# Autodesk Inventor assembly: Baugruppe1
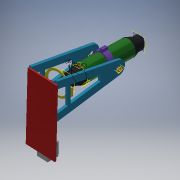
[picture p0: Inventor's stored thumbnail of the model, 180x180]
Saved by Autodesk Inventor 2017 (Build 210142000, 142)
## iProperties
Part Number: Baugruppe1
Material: Generisch
Document SubType Name: Assembly
Designer: Fabio
Author: Fabio
## Documents named in this file (10)
- C:\Users\Fabio\dicer\inventor\Baugruppe1.iam
- C:\Users\Fabio\dicer\inventor\cylinder.ipt
- C:\Users\Fabio\dicer\inventor\endkappen.ipt
- C:\Users\Fabio\dicer\inventor\spannringe.ipt
- C:\Users\Fabio\dicer\inventor\kamera_dummy.ipt
- C:\Users\Fabio\dicer\inventor\spannring_achse.ipt
- C:\Users\Fabio\dicer\inventor\halter_seite.ipt
- C:\Users\Fabio\dicer\inventor\grundplatte.ipt
- C:\Users\Fabio\dicer\inventor\LED_Ring.ipt
- C:\Users\Fabio\dicer\inventor\spiegelhalter.ipt
## Components (13 placed, 9 different names)
1. cylinder:1 — Passend:1, Passend:3, Einfügen:1, Einfügen:2, Passend:5
2. endkappen:1 — Passend:1
3. endkappen:2 — Passend:5
4. kamera_dummy:1 — Passend:4
5. spannringe:1 — Einfügen:1, Einfügen:4
6. spannringe:2 — Passend:3, Einfügen:2, Einfügen:7
7. spannring_achse:2 — Einfügen:4, Einfügen:6
8. halter_seite:1 — Einfügen:6
9. grundplatte:1 — Passend:4, Einfügen:9
10. LED_Ring:1 — Passend:6
11. spannring_achse:3 — Einfügen:7, Einfügen:8
12. halter_seite:2 — Einfügen:8, Einfügen:9, Passend:6
13. spiegelhalter:1
## Relationships (12: Insert 7, Mate 5)
- Passend:1 [Mate]: cylinder:1 ↔ endkappen:1
- Passend:3 [Mate]: cylinder:1 ↔ spannringe:2
- Einfügen:1 [Insert] (-100 mm): cylinder:1 ↔ spannringe:1
- Einfügen:2 [Insert] (-100 mm): cylinder:1 ↔ spannringe:2
- Einfügen:4 [Insert]: spannringe:1 ↔ spannring_achse:2
- Einfügen:6 [Insert] (10 mm): spannring_achse:2 ↔ halter_seite:1
- Passend:4 [Mate]: kamera_dummy:1 ↔ grundplatte:1
- Passend:5 [Mate]: cylinder:1 ↔ endkappen:2
- Einfügen:7 [Insert]: spannringe:2 ↔ spannring_achse:3
- Einfügen:8 [Insert] (-20 mm): spannring_achse:3 ↔ halter_seite:2
- Einfügen:9 [Insert]: grundplatte:1 ↔ halter_seite:2
- Passend:6 [Mate]: LED_Ring:1 ↔ halter_seite:2
